# Autodesk Inventor assembly: FemaleHeader-02
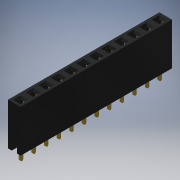
[picture p0: Inventor's stored thumbnail of the model, 180x180]
Saved by Autodesk Inventor 2018 (Build 220112000, 112)
## iProperties
Created: 2013-05-21
Part Number: FemaleHeader-02
Document SubType Name: Assembly
Designer: dkt01
Sending System: SolidWorks 2012
Last Author: simonx
Last Saved: 2013-05-21
pinx: 1.000 ul
piny: 12.000 ul
Author: dkt01
## Documents named in this file (2)
- C:\Users\dktur\Dropbox\StackLightMonitor\CAD\FemaleHeader-02.iam
- C:\Users\dktur\Dropbox\StackLightMonitor\CAD\FemaleHeader_Single-02.iam
## Components (12 placed, 2 different names)
1. header:1 [sub-assembly]
2. FemaleHeader_Single-02:5 [sub-assembly]
3. FemaleHeader_Single-02:6 [sub-assembly]
4. FemaleHeader_Single-02:7 [sub-assembly]
5. FemaleHeader_Single-02:8 [sub-assembly]
6. FemaleHeader_Single-02:9 [sub-assembly]
7. FemaleHeader_Single-02:10 [sub-assembly]
8. FemaleHeader_Single-02:11 [sub-assembly]
9. FemaleHeader_Single-02:12 [sub-assembly]
10. FemaleHeader_Single-02:13 [sub-assembly]
11. FemaleHeader_Single-02:14 [sub-assembly]
12. FemaleHeader_Single-02:15 [sub-assembly]
## Component patterns: (12 elements, first: header:1)
